# Autodesk Inventor assembly: Health_module_ucBoard
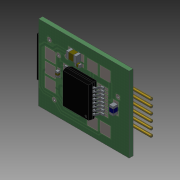
[picture p0: Inventor's stored thumbnail of the model, 180x180]
Saved by Autodesk Inventor 2013 (Build 170138000, 138)
## iProperties
Created: 2015-07-04
Part Number: Health_module_ucBoard
Document SubType Name: Assembly
Designer: terg
Author: terg
## Documents named in this file (10)
- C:\Users\terg\Projects\ModularElectronics\3D_models\Health_module\Health_module_ucBoard.iam
- C:\Users\terg\Projects\ModularElectronics\3D_models\Health_module\Health_module_uCBoard.ipt
- C:\Users\terg\Projects\ModularElectronics\3D_models\Components\0805_cap.ipt
- C:\Users\terg\Projects\ModularElectronics\3D_models\Components\0402_cap.ipt
- C:\Users\terg\Projects\ModularElectronics\3D_models\Components\0603_res.ipt
- C:\Users\terg\Projects\ModularElectronics\3D_models\Components\0402_res.ipt
- C:\Users\terg\Projects\ModularElectronics\3D_models\Components\EFM32ZG110.ipt
- C:\Users\terg\Projects\ModularElectronics\3D_models\Health_module\AD5933.ipt
- C:\Users\terg\Projects\ModularElectronics\3D_models\Components\FemalConnector.ipt
- C:\Users\terg\Projects\ModularElectronics\3D_models\Components\MaleConnector.ipt
## Components (18 placed, 9 different names)
1. Health_module_uCBoard:1 — Zestawiający:1, Zestawiający:2, Zestawiający:3, Równoległy:1, Równoległy:2, Równoległy:3, Równoległy:4, Równoległy:5, Równoległy:6, Zestawiający:4, Równoległy:7, Równoległy:8, Zestawiający:5, Zestawiający:6, Zestawiający:7, Zestawiający:10, Zestawiający:11, Zestawiający:12, Zestawiający:13, Równoległy:9, Równoległy:10, Równoległy:11, Równoległy:12, Równoległy:13, Równoległy:14, Równoległy:15, Równoległy:16, Równoległy:17, Równoległy:18, Równoległy:19, Równoległy:20, Równoległy:21, Równoległy:22, Zestawiający:14, Zestawiający:15, Równoległy:23, Równoległy:24, Równoległy:25, Równoległy:26, Zestawiający:16, Równoległy:27, Równoległy:28, Zestawiający:17, Równoległy:29, Równoległy:30, Zestawiający:18, Zestawiający:19, Równoległy:31, Równoległy:32, Równoległy:33, Równoległy:34
2. 0805_cap:1 — Zestawiający:1, Równoległy:1, Równoległy:4
3. 0402_cap:1 — Zestawiający:2, Równoległy:2, Równoległy:5
4. 0402_cap:2 — Zestawiający:3, Równoległy:3, Równoległy:6
5. 0603_res:1 — Zestawiający:4, Równoległy:7, Równoległy:8
6. 0402_cap:3 — Zestawiający:5, Równoległy:10, Równoległy:14
7. 0402_cap:4 — Zestawiający:6, Równoległy:11, Równoległy:15
8. 0402_cap:5 — Zestawiający:7, Równoległy:12, Równoległy:16
9. 0402_cap:8 — Zestawiający:12, Równoległy:19, Równoległy:22
10. 0402_res:1 — Zestawiający:10, Równoległy:9, Równoległy:13
11. 0402_res:2 — Zestawiający:11, Równoległy:17, Równoległy:21
12. 0402_res:3 — Zestawiający:13, Równoległy:18, Równoległy:20
13. 0805_cap:2 — Zestawiający:14, Równoległy:23, Równoległy:24
14. 0805_cap:3 — Zestawiający:15, Równoległy:25, Równoległy:26
15. EFM32ZG110:1 — Zestawiający:16, Równoległy:27, Równoległy:28
16. AD5933:1 — Zestawiający:17, Równoległy:29, Równoległy:30
17. FemalConnector:1 — Zestawiający:18, Równoległy:31, Równoległy:32
18. MaleConnector:1 — Zestawiający:19, Równoległy:33, Równoległy:34
## Relationships (51: Flush 34, Mate 17)
- Zestawiający:1 [Mate]: Health_module_uCBoard:1 ↔ 0805_cap:1
- Zestawiający:2 [Mate]: Health_module_uCBoard:1 ↔ 0402_cap:1
- Zestawiający:3 [Mate]: Health_module_uCBoard:1 ↔ 0402_cap:2
- Równoległy:1 [Flush] (6.424 mm): Health_module_uCBoard:1 ↔ 0805_cap:1
- Równoległy:2 [Flush] (7.668 mm): Health_module_uCBoard:1 ↔ 0402_cap:1
- Równoległy:3 [Flush] (3.801 mm): Health_module_uCBoard:1 ↔ 0402_cap:2
- Równoległy:4 [Flush] (1.777 mm): Health_module_uCBoard:1 ↔ 0805_cap:1
- Równoległy:5 [Flush] (3.453 mm): Health_module_uCBoard:1 ↔ 0402_cap:1
- Równoległy:6 [Flush] (6.767 mm): Health_module_uCBoard:1 ↔ 0402_cap:2
- Zestawiający:4 [Mate]: Health_module_uCBoard:1 ↔ 0603_res:1
- Równoległy:7 [Flush] (2.249 mm): Health_module_uCBoard:1 ↔ 0603_res:1
- Równoległy:8 [Flush] (6.852 mm): Health_module_uCBoard:1 ↔ 0603_res:1
- Zestawiający:5 [Mate]: Health_module_uCBoard:1 ↔ 0402_cap:3
- Zestawiający:6 [Mate]: Health_module_uCBoard:1 ↔ 0402_cap:4
- Zestawiający:7 [Mate]: Health_module_uCBoard:1 ↔ 0402_cap:5
- Zestawiający:10 [Mate]: Health_module_uCBoard:1 ↔ 0402_res:1
- Zestawiający:11 [Mate]: Health_module_uCBoard:1 ↔ 0402_res:2
- Zestawiający:12 [Mate]: Health_module_uCBoard:1 ↔ 0402_cap:8
- Zestawiający:13 [Mate]: Health_module_uCBoard:1 ↔ 0402_res:3
- Równoległy:9 [Flush] (2.624 mm): Health_module_uCBoard:1 ↔ 0402_res:1
- Równoległy:10 [Flush] (2.889 mm): Health_module_uCBoard:1 ↔ 0402_cap:3
- Równoległy:11 [Flush] (3.792 mm): Health_module_uCBoard:1 ↔ 0402_cap:4
- Równoległy:12 [Flush] (7.086 mm): Health_module_uCBoard:1 ↔ 0402_cap:5
- Równoległy:13 [Flush] (5.359 mm): Health_module_uCBoard:1 ↔ 0402_res:1
- Równoległy:14 [Flush] (8.889 mm): Health_module_uCBoard:1 ↔ 0402_cap:3
- Równoległy:15 [Flush] (9.968 mm): Health_module_uCBoard:1 ↔ 0402_cap:4
- Równoległy:16 [Flush] (13.023 mm): Health_module_uCBoard:1 ↔ 0402_cap:5
- Równoległy:17 [Flush] (5.275 mm): Health_module_uCBoard:1 ↔ 0402_res:2
- Równoległy:18 [Flush] (5.302 mm): Health_module_uCBoard:1 ↔ 0402_res:3
- Równoległy:19 [Flush] (8.581 mm): Health_module_uCBoard:1 ↔ 0402_cap:8
- Równoległy:20 [Flush] (2.92 mm): Health_module_uCBoard:1 ↔ 0402_res:3
- Równoległy:21 [Flush] (3.968 mm): Health_module_uCBoard:1 ↔ 0402_res:2
- Równoległy:22 [Flush] (2.668 mm): Health_module_uCBoard:1 ↔ 0402_cap:8
- Zestawiający:14 [Mate]: Health_module_uCBoard:1 ↔ 0805_cap:2
- Zestawiający:15 [Mate]: Health_module_uCBoard:1 ↔ 0805_cap:3
- Równoległy:23 [Flush] (4.073 mm): Health_module_uCBoard:1 ↔ 0805_cap:2
- Równoległy:24 [Flush] (8.531 mm): Health_module_uCBoard:1 ↔ 0805_cap:2
- Równoległy:25 [Flush] (13.9 mm): Health_module_uCBoard:1 ↔ 0805_cap:3
- Równoległy:26 [Flush] (1.89 mm): Health_module_uCBoard:1 ↔ 0805_cap:3
- Zestawiający:16 [Mate]: Health_module_uCBoard:1 ↔ EFM32ZG110:1
- Równoległy:27 [Flush] (4.847 mm): Health_module_uCBoard:1 ↔ EFM32ZG110:1
- Równoległy:28 [Flush] (6.343 mm): Health_module_uCBoard:1 ↔ EFM32ZG110:1
- Zestawiający:17 [Mate]: Health_module_uCBoard:1 ↔ AD5933:1
- Równoległy:29 [Flush] (4.829 mm): Health_module_uCBoard:1 ↔ AD5933:1
- Równoległy:30 [Flush] (4.229 mm): Health_module_uCBoard:1 ↔ AD5933:1
- Zestawiający:18 [Mate]: Health_module_uCBoard:1 ↔ FemalConnector:1
- Zestawiający:19 [Mate]: Health_module_uCBoard:1 ↔ MaleConnector:1
- Równoległy:31 [Flush] (3.578 mm): Health_module_uCBoard:1 ↔ FemalConnector:1
- Równoległy:32 [Flush] (1.171 mm): Health_module_uCBoard:1 ↔ FemalConnector:1
- Równoległy:33 [Flush] (-4.104 mm): Health_module_uCBoard:1 ↔ MaleConnector:1
- Równoległy:34 [Flush] (2.914 mm): Health_module_uCBoard:1 ↔ MaleConnector:1
